# Autodesk Inventor assembly: Bearing_ASM
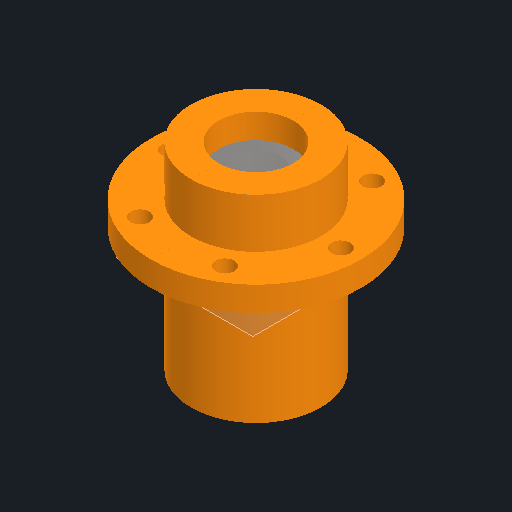
[picture p0: Inventor's stored thumbnail of the model, 512x512]
Saved by Autodesk Inventor 2024.1 (Build 281209000, 209)
## iProperties
Created: 2023-08-04
Part Number: Bearing_ASM
Document SubType Name: Assembly
Designer: jaege
Author: jaege
## Documents named in this file (3)
- C:\Users\jaege\VUB\Schakel_Ind_Elo\Year_1_Both\BA_Thesis\3D_Files\Lift_V2\Bearing_ASM.iam
- C:\Users\jaege\VUB\Schakel_Ind_Elo\Year_1_Both\BA_Thesis\3D_Files\Lift_V2\Bearing_Holder.ipt
- C:\Users\jaege\VUB\Schakel_Ind_Elo\Year_1_Both\BA_Thesis\3D_Files\Lift_V2\LinearBearing.ipt
## Components (3 placed, 2 different names)
1. Bearing_Holder:1
2. LinearBearing:1
3. Bearing_Holder:2
## Relationships (5: Mate 5)
- [Mate]: Bearing_Holder:1 ↔ LinearBearing:1
- [Mate]: Bearing_Holder:1 ↔ LinearBearing:1
- [Mate]: Bearing_Holder:1 ↔ Bearing_Holder:2
- [Mate]: LinearBearing:1 ↔ Bearing_Holder:2
- [Mate]: LinearBearing:1 ↔ Bearing_Holder:2
